# Autodesk Inventor assembly: frEonV2-OP3t
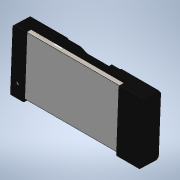
[picture p0: Inventor's stored thumbnail of the model, 180x180]
Saved by Autodesk Inventor 2020 (Build 240168000, 168)
## iProperties
Created: 2021-07-02
Part Number: frEonV2-OP3t
Document SubType Name: Assembly
Designer: dkiiv
Author: dkiiv
## Documents named in this file (4)
- D:\CAD\leeco-freon\V2\frEonV2-OP3t.iam
- D:\CAD\leeco-freon\V2\printed parts\rightOP3t.ipt
- D:\CAD\leeco-freon\V2\printed parts\leftOP3t.ipt
- D:\CAD\leeco-freon\V2\OnePlus3Tproper.ipt
## Components (3 placed, 3 different names)
1. rightOP3t:1 — Flush:1, Flush:2, Mate:4
2. leftOP3t:1 — Flush:1, Flush:2, Mate:1, Mate:2, Mate:3
3. OnePlus3Tproper:1 — Mate:1, Mate:2, Mate:3, Mate:4
## Relationships (6: Mate 4, Flush 2)
- Flush:1: rightOP3t:1 ↔ leftOP3t:1
- Flush:2: rightOP3t:1 ↔ leftOP3t:1
- Mate:1: leftOP3t:1 ↔ OnePlus3Tproper:1
- Mate:2: leftOP3t:1 ↔ OnePlus3Tproper:1
- Mate:3: leftOP3t:1 ↔ OnePlus3Tproper:1
- Mate:4: rightOP3t:1 ↔ OnePlus3Tproper:1
